# Autodesk Inventor assembly: wheel
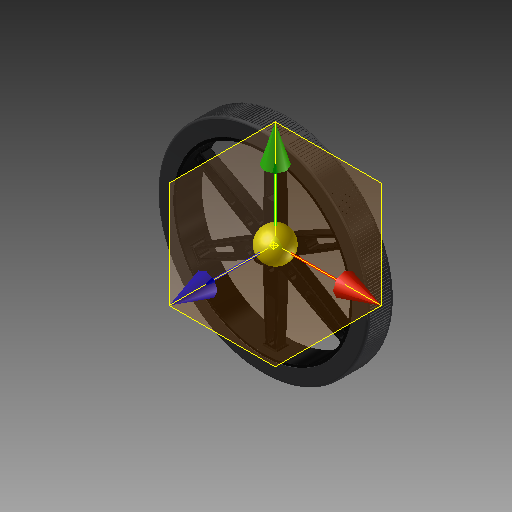
[picture p0: Inventor's stored thumbnail of the model, 512x512]
Saved by Autodesk Inventor 2018 (Build 220112000, 112)
## iProperties
Created: 2019-05-16
Part Number: wheel
Material: 一般
Document SubType Name: Assembly
Designer: ku_sk
Mass: 19.7 g
Surface Area: 203.788 cm^2
Volume: 18.5895 cm^3
Density: 1.05974 g/cm^3
Sending System: Autodesk Inventor 2018
OS: Windows
FORMAT: text
GUISE: transmit
KEY: wheel
FILE: D:\windows\InventorProjects\Balboa32U4\parts\wheel.x_t
DATE: 2019-May-16 18:05:34
Author: ku_sk
## Documents named in this file (3)
- D:\Inventor\Balboa32U4-CAD\parts\wheel\wheelR80.iam
- D:\Inventor\Balboa32U4-CAD\parts\wheel\parts\tyre.ipt
- D:\Inventor\Balboa32U4-CAD\parts\wheel\parts\wheel.ipt
## Components (2 placed, 2 different names)
1. tyre — メイト:7, メイト:9
2. wheel — メイト:6, メイト:7, メイト:8, メイト:9, 角度:1
## Relationships (5: Mate 4, Angle 1)
- メイト:6 [Mate]: wheel
- メイト:7 [Mate]: tyre ↔ wheel
- メイト:8 [Mate]: wheel
- メイト:9 [Mate]: tyre ↔ wheel
- 角度:1 [Angle] (0 deg): wheel
